# Autodesk Inventor assembly: Wheel Bearing 1764
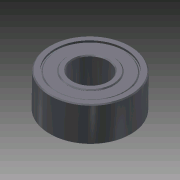
[picture p0: Inventor's stored thumbnail of the model, 180x180]
Saved by Autodesk Inventor 2011 (Build 150239000, 239)
## iProperties
Created: 2009-01-08
Part Number: Wheel Bearing 1764
Document SubType Name: Assembly
Designer: pmulligan
Author: pmulligan
## Documents named in this file (3)
- R:\CAD Archives\Wheels\Wheel Bearing 1764\Wheel Bearing 1764.iam
- R:\CAD Archives\Wheels\Wheel Bearing 1764\Outer Casing 1764.ipt
- R:\CAD Archives\Wheels\Wheel Bearing 1764\Inner Ring 1764.ipt
## Components (2 placed, 2 different names)
1. Outer Casing 1764:1 — Mate:1, Mate:2
2. Inner Ring 1764:1 — Mate:1, Mate:2, Angle:1, Mate:4
## Relationships (4: Mate 3, Angle 1)
- Mate:1: Outer Casing 1764:1 ↔ Inner Ring 1764:1
- Mate:2: Outer Casing 1764:1 ↔ Inner Ring 1764:1
- Angle:1 (0 deg): Inner Ring 1764:1
- Mate:4: Inner Ring 1764:1
